# Autodesk Inventor assembly: SistemaDeElevación
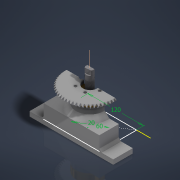
[picture p0: Inventor's stored thumbnail of the model, 180x180]
Saved by Autodesk Inventor 2022 (Build 260153000, 153)
## iProperties
Created: 2021-09-10
Part Number: SistemaDeElevación
Material: Generic
Document SubType Name: Assembly
Designer: Andres
Author: Andres
## Documents named in this file (6)
- D:\Documentos\15.PUCP_2021-2\[PDM] Proyecto de Diseño Mecatrónico\RobotPallet\SistemaDeElevación.iam
- D:\Documentos\15.PUCP_2021-2\[PDM] Proyecto de Diseño Mecatrónico\RobotPallet\soporte de rodamientos.ipt
- D:\Documentos\15.PUCP_2021-2\[PDM] Proyecto de Diseño Mecatrónico\RobotPallet\Tuerca.ipt
- D:\Documentos\15.PUCP_2021-2\[PDM] Proyecto de Diseño Mecatrónico\RobotPallet\SistemaDeElevación\Design Accelerator\Bearing1.iam
- D:\Documentos\15.PUCP_2021-2\[PDM] Proyecto de Diseño Mecatrónico\RobotPallet\Tornillo de elevación.ipt
- D:\Documentos\15.PUCP_2021-2\[PDM] Proyecto de Diseño Mecatrónico\RobotPallet\SistemaDeElevación\Design Accelerator\Bevel Gears1.iam
## Components (5 placed, 5 different names)
1. soporte de rodamientos:1 — Mate:1, Mate:2
2. Tuerca:1 — Mate:3, Mate:4, Cylindrical:1, Mate:5, Angle:1
3. Bearing:1 [sub-assembly] — Mate:1, Mate:2, Mate:3, Mate:4
4. Tornillo de elevación:1 — Cylindrical:1
5. Bevel Gears:1 [sub-assembly] — Mate:5, Angle:1
## Relationships (7: Mate 5, CylindricalJoint 1, Angle 1)
- Mate:1: soporte de rodamientos:1 ↔ Bearing:1
- Mate:2: soporte de rodamientos:1 ↔ Bearing:1
- Mate:3: Tuerca:1 ↔ Bearing:1
- Mate:4: Tuerca:1 ↔ Bearing:1
- Cylindrical:1: Tuerca:1 ↔ Tornillo de elevación:1
- Mate:5: Tuerca:1 ↔ Bevel Gears:1
- Angle:1 (0 deg): Tuerca:1 ↔ Bevel Gears:1
